# Autodesk Inventor assembly: CompleteModuleHolderMid
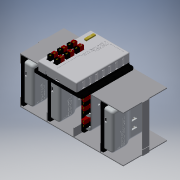
[picture p0: Inventor's stored thumbnail of the model, 180x180]
Saved by Autodesk Inventor 2016 (Build 200138000, 138)
## iProperties
Created: 2016-11-16
Part Number: CompleteModuleHolderMid
Document SubType Name: Assembly
Designer: RoboticsUser
Author: RoboticsUser
## Documents named in this file (5)
- C:\Robotics\CAD\2016-17_CAD\CompleteModuleHolderMid.iam
- C:\Robotics\CAD\2016-17_CAD\ModulePlate2.0.ipt
- C:\Robotics\CAD\2016-17_CAD\ModulePlate2.0Top.ipt
- C:\Robotics\CAD\COTSParts\ModernRobotics\MRI45-2203_Motor_Controller.ipt
- C:\Robotics\CAD\COTSParts\ModernRobotics\MRI45-2200_Power_Distribution_Module.ipt
## Components (7 placed, 4 different names)
1. ModulePlate2.0:1 — Mate:3, Mate:4, Flush:2, Mate:5, Mate:6, Flush:3, Mate:7, Mate:8, Flush:4, Flush:5, Flush:6, Mate:10, Mate:11
2. ModulePlate2.0Top:1 — Mate:9, Flush:5, Flush:6, Flush:7, Mate:12, Flush:8, Flush:9
3. MRI45-2203_Motor_Controller:1 — Mate:10, Mate:11, Flush:7
4. MRI45-2203_Motor_Controller:2 — Mate:5, Mate:6, Flush:3, Mate:9
5. MRI45-2203_Motor_Controller:3 — Mate:7, Mate:8, Flush:4
6. MRI45-2203_Motor_Controller:4 — Mate:3, Mate:4, Flush:2
7. MRI45-2200_Power_Distribution_Module:1 — Mate:12, Flush:8, Flush:9
## Relationships (18: Mate 10, Flush 8)
- Mate:3: ModulePlate2.0:1 ↔ MRI45-2203_Motor_Controller:4
- Mate:4: ModulePlate2.0:1 ↔ MRI45-2203_Motor_Controller:4
- Flush:2: ModulePlate2.0:1 ↔ MRI45-2203_Motor_Controller:4
- Mate:5: ModulePlate2.0:1 ↔ MRI45-2203_Motor_Controller:2
- Mate:6: ModulePlate2.0:1 ↔ MRI45-2203_Motor_Controller:2
- Flush:3: ModulePlate2.0:1 ↔ MRI45-2203_Motor_Controller:2
- Mate:7: ModulePlate2.0:1 ↔ MRI45-2203_Motor_Controller:3
- Mate:8: ModulePlate2.0:1 ↔ MRI45-2203_Motor_Controller:3
- Flush:4: ModulePlate2.0:1 ↔ MRI45-2203_Motor_Controller:3
- Mate:9: ModulePlate2.0Top:1 ↔ MRI45-2203_Motor_Controller:2
- Flush:5: ModulePlate2.0:1 ↔ ModulePlate2.0Top:1
- Flush:6: ModulePlate2.0:1 ↔ ModulePlate2.0Top:1
- Mate:10: ModulePlate2.0:1 ↔ MRI45-2203_Motor_Controller:1
- Mate:11: ModulePlate2.0:1 ↔ MRI45-2203_Motor_Controller:1
- Flush:7: ModulePlate2.0Top:1 ↔ MRI45-2203_Motor_Controller:1
- Mate:12: ModulePlate2.0Top:1 ↔ MRI45-2200_Power_Distribution_Module:1
- Flush:8: ModulePlate2.0Top:1 ↔ MRI45-2200_Power_Distribution_Module:1
- Flush:9 (63.5 mm): ModulePlate2.0Top:1 ↔ MRI45-2200_Power_Distribution_Module:1
